# Autodesk Inventor assembly: Joint Assembly
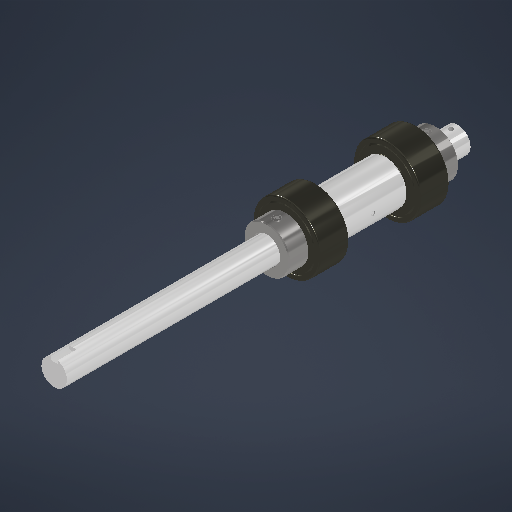
[picture p0: Inventor's stored thumbnail of the model, 512x512]
Saved by Autodesk Inventor 2026.3 (Build 303398000, 398)
## iProperties
Created: 2026-07-22
Part Number: Joint Assembly
Document SubType Name: Assembly
Designer: matot
Author: matot
## Documents named in this file (4)
- C:\Users\matot\OneDrive - Stellenbosch University\2026\MechatronicsProject478\Building the joint\Joint Assembly\Joint Assembly.iam
- C:\Users\matot\OneDrive - Stellenbosch University\2026\MechatronicsProject478\Building the joint\Joint Assembly\Final joint shaft.ipt
- C:\Users\matot\OneDrive - Stellenbosch University\2026\MechatronicsProject478\Building the joint\Joint Assembly\2058786.iam
- C:\Users\matot\OneDrive - Stellenbosch University\2026\MechatronicsProject478\Building the joint\Joint Assembly\8236967.ipt
## Components (5 placed, 3 different names)
1. Final joint shaft:1 — Insert:1, Insert:2
2. 2058786:1 [sub-assembly] — Insert:2, Insert:4
3. 2058786:2 [sub-assembly] — Insert:1, Insert:3
4. 8236967:1 — Insert:4
5. 8236967:2 — Insert:3
## Relationships (4: Insert 4)
- Insert:1: Final joint shaft:1 ↔ 2058786:2
- Insert:2: Final joint shaft:1 ↔ 2058786:1
- Insert:3: 2058786:2 ↔ 8236967:2
- Insert:4: 2058786:1 ↔ 8236967:1
